# Autodesk Inventor assembly: rev6
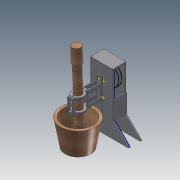
[picture p0: Inventor's stored thumbnail of the model, 180x180]
Saved by Autodesk Inventor 2015 (Build 190159000, 159)
## iProperties
Created: 2014-08-31
Part Number: rev6
Document SubType Name: Assembly
Designer: shohei
Author: shohei
## Documents named in this file (28)
- C:\Users\shohei\Documents\Inventor\FufuPounderGeared\rev6.iam
- C:\Users\shohei\Documents\Inventor\FufuPounderGeared\mortar2.ipt
- C:\Users\shohei\Documents\Inventor\FufuPounderGeared\sideplate.ipt
- C:\Users\shohei\Documents\Inventor\FufuPounderGeared\mainpulley.ipt
- C:\Users\shohei\Documents\Inventor\FufuPounderGeared\shaft5.ipt
- C:\Users\shohei\Documents\Inventor\FufuPounderGeared\drivelever.ipt
- C:\Users\shohei\Documents\Inventor\FufuPounderGeared\shaft7.ipt
- C:\Users\shohei\Documents\Inventor\FufuPounderGeared\globals.ipt
- C:\Users\shohei\Documents\Inventor\FufuPounderGeared\shaft8.ipt
- C:\Users\shohei\Documents\Inventor\FufuPounderGeared\shaft9.ipt
- C:\Users\shohei\Documents\Inventor\FufuPounderGeared\mallet_new.ipt
- C:\Users\shohei\Documents\Inventor\FufuPounderGeared\mallet_holder.ipt
- C:\Users\shohei\Documents\Inventor\FufuPounderGeared\mallet_sideplate.ipt
- C:\Users\shohei\Documents\Inventor\FufuPounderGeared\holderBlock.ipt
- C:\Users\shohei\Documents\Inventor\FufuPounderGeared\sideplate_top.ipt
- C:\Users\shohei\Documents\Inventor\FufuPounderGeared\shaft10.ipt
- C:\Users\shohei\Documents\Inventor\FufuPounderGeared\holderBlock2.ipt
- C:\Users\shohei\Documents\Inventor\FufuPounderGeared\gripsupport.ipt
- C:\Users\shohei\Documents\Inventor\FufuPounderGeared\M10washer.ipt
- C:\Users\shohei\Documents\Inventor\FufuPounderGeared\pulleyFlange.ipt
- C:\Users\shohei\Documents\Inventor\FufuPounderGeared\guardplate.ipt
- C:\Users\shohei\Documents\Inventor\FufuPounderGeared\drivepulleyAssembly.iam
- C:\Users\shohei\Documents\Inventor\FufuPounder\rev6\AIP\FEA\b5u4ebwdc.fins
- C:\Users\shohei\Documents\Inventor\FufuPounder\rev6\AIP\FEA\b5u4ebwdc.fsat
- C:\Users\shohei\Documents\Inventor\FufuPounder\rev6\AIP\FEA\b5u4ebwdc.ftes
- C:\Users\shohei\Documents\Inventor\FufuPounder\rev6\AIP\FEA\b5u4ebwdc.fwiz
- C:\Users\shohei\Documents\Inventor\FufuPounder\rev6\AIP\FEA\b5u4ebwgw.fmsh
- C:\Users\shohei\Documents\Inventor\FufuPounder\rev6\AIP\FEA\b5u4ebwgx.fres
## Components (46 placed, 21 different names)
1. mortar2:1 — Mate:1
2. sideplate:1 — Mate:2, Flush:1, Slider:1, Mate:9, Flush:13, Flush:14, Rotational:17, Flush:41, Mate:22
3. sideplate:2 — Mate:3, Flush:1, Rotational:10, Flush:15, Slider:2, Rotational:31, Mate:21, Flush:42
4. mainpulley:1 — Angle:1, Rotational:32, Cylindrical:6, Rigid:36, Rigid:38
5. shaft5:2 — Rotational:8, Cylindrical:6, Cylindrical:7
6. drivelever:1 — Cylindrical:1, Rotational:8, Rotational:23, Rotational:24, Rotational:25, Rotational:26
7. shaft7:1 — Slider:1, Cylindrical:1, Rotational:14, Rotational:18, Rotational:19, Rotational:20, Rotational:21
8. globals:1
9. mainpulley:2 — Cylindrical:7, Rotational:33, Rigid:35, Rigid:37
10. shaft8:1 — Rotational:10, Rotational:33
11. shaft9:2 — Cylindrical:4, Cylindrical:5, Slider:2, Rigid:2, Rotational:22
12. mallet_new:1 — Rigid:1
13. mallet_holder:1 — Flush:3, Mate:5, Flush:4, Mate:6, Flush:5, Flush:6, Flush:9, Mate:7, Flush:10, Mate:8, Flush:11, Flush:12, Rigid:1, Flush:32
14. mallet_holder:2 — Flush:7, Mate:15, Flush:29, Flush:37
15. mallet_sideplate:1 — Flush:3, Mate:5, Flush:4, Flush:7, Mate:15, Flush:34, Flush:35, Mate:18, Mate:19, Flush:38, Flush:39
16. mallet_sideplate:2 — Flush:9, Mate:7, Flush:10
17. mallet_sideplate:3 — Mate:6, Flush:5, Flush:6, Mate:16, Mate:17, Flush:33, Flush:36
18. mallet_sideplate:4 — Mate:8, Flush:11, Flush:12, Flush:37
19. holderBlock:2 — Rotational:14, Cylindrical:4
20. sideplate_top:1 — Mate:9, Flush:13, Flush:14, Flush:15
21. shaft10:1 — Rotational:17, Rotational:30, Rotational:32, Insert:1
22. holderBlock2:1 — Rotational:18, Cylindrical:5, Flush:28, Flush:40, Mate:20
23. gripsupport:1 — Flush:32, Mate:17, Flush:33, Flush:40
24. gripsupport:2 — Flush:34, Flush:35, Mate:18, Mate:20
25. gripsupport:3 — Mate:19, Flush:38, Flush:39
26. gripsupport:4 — Mate:16, Flush:28, Flush:29, Flush:36
27. pulleyFlange:1 — Rigid:36
28. pulleyFlange:2
29. pulleyFlange:3 — Rigid:35
30. guardplate:1 — Mate:22, Flush:42
31. guardplate:2 — Mate:21, Flush:41
32. drivepulleyAssembly:1 [sub-assembly] — Insert:1
33. M10washer:1 — Rigid:37
34. M10washer:2 — Rotational:19
35. M10washer:3 — Rotational:24
36. M10washer:4 — Rotational:25
37. M10washer:5 — Rotational:21
38. M10washer:6 — Rotational:22
39. M10washer:7 — Rotational:26
40. M10washer:8 — Rotational:23
41. M10washer:9 — Rotational:20
42. M10washer:10 — Rigid:2
43. M10washer:11 — Rigid:38
44. M10washer:14 — Rotational:31
45. M10washer:18 — Rotational:30
46. M10washer:22
## Relationships (74: Flush 26, RevoluteJoint 17, Mate 16, WeldJoint 6, CylindricalJoint 5, TranslationJoint 2, Angle 1, Insert 1)
- Mate:1: mortar2:1
- Mate:2: sideplate:1
- Mate:3: sideplate:2
- Flush:1: sideplate:1 ↔ sideplate:2
- Slider:1 [TranslationJoint]: sideplate:1 ↔ shaft7:1
- Cylindrical:1: drivelever:1 ↔ shaft7:1
- Rotational:8 [RevoluteJoint] (-30 mm): shaft5:2 ↔ drivelever:1
- Angle:1 (51.6389 deg): mainpulley:1
- Rotational:10 [RevoluteJoint]: sideplate:2 ↔ shaft8:1
- Flush:3: mallet_holder:1 ↔ mallet_sideplate:1
- Mate:5: mallet_holder:1 ↔ mallet_sideplate:1
- Flush:4: mallet_holder:1 ↔ mallet_sideplate:1
- Mate:6: mallet_holder:1 ↔ mallet_sideplate:3
- Flush:5: mallet_holder:1 ↔ mallet_sideplate:3
- Flush:6: mallet_holder:1 ↔ mallet_sideplate:3
- Flush:7: mallet_holder:2 ↔ mallet_sideplate:1
- Flush:9: mallet_holder:1 ↔ mallet_sideplate:2
- Mate:7: mallet_holder:1 ↔ mallet_sideplate:2
- Flush:10: mallet_holder:1 ↔ mallet_sideplate:2
- Mate:8: mallet_holder:1 ↔ mallet_sideplate:4
- Flush:11: mallet_holder:1 ↔ mallet_sideplate:4
- Flush:12: mallet_holder:1 ↔ mallet_sideplate:4
- Rotational:14 [RevoluteJoint] (-30 mm): shaft7:1 ↔ holderBlock:2
- Cylindrical:4: shaft9:2 ↔ holderBlock:2
- Mate:9: sideplate:1 ↔ sideplate_top:1
- Flush:13: sideplate:1 ↔ sideplate_top:1
- Flush:14: sideplate:1 ↔ sideplate_top:1
- Flush:15: sideplate:2 ↔ sideplate_top:1
- Rotational:17 [RevoluteJoint] (-80 mm): sideplate:1 ↔ shaft10:1
- Rotational:18 [RevoluteJoint]: shaft7:1 ↔ holderBlock2:1
- Cylindrical:5: shaft9:2 ↔ holderBlock2:1
- Mate:15: mallet_holder:2 ↔ mallet_sideplate:1
- Rigid:1 [WeldJoint]: mallet_new:1 ↔ mallet_holder:1
- Slider:2 [TranslationJoint]: sideplate:2 ↔ shaft9:2
- Mate:16: mallet_sideplate:3 ↔ gripsupport:4
- Flush:28: holderBlock2:1 ↔ gripsupport:4
- Flush:29: mallet_holder:2 ↔ gripsupport:4
- Rotational:19 [RevoluteJoint] (-22 mm): shaft7:1 ↔ M10washer:2
- Rotational:20 [RevoluteJoint] (-50 mm): shaft7:1 ↔ M10washer:9
- Rigid:2 [WeldJoint] (-20 mm): shaft9:2 ↔ M10washer:10
- Rotational:21 [RevoluteJoint] (-30 mm): shaft7:1 ↔ M10washer:5
- Rotational:22 [RevoluteJoint]: shaft9:2 ↔ M10washer:6
- Rotational:23 [RevoluteJoint] (-2 mm): drivelever:1 ↔ M10washer:8
- Rotational:24 [RevoluteJoint]: drivelever:1 ↔ M10washer:3
- Rotational:25 [RevoluteJoint]: drivelever:1 ↔ M10washer:4
- Rotational:26 [RevoluteJoint]: drivelever:1 ↔ M10washer:7
- Rotational:30 [RevoluteJoint] (-10 mm): shaft10:1 ↔ M10washer:18
- Rotational:31 [RevoluteJoint] (-2 mm): sideplate:2 ↔ M10washer:14
- Rotational:32 [RevoluteJoint]: mainpulley:1 ↔ shaft10:1
- Cylindrical:6: mainpulley:1 ↔ shaft5:2
- Cylindrical:7: shaft5:2 ↔ mainpulley:2
- Rotational:33 [RevoluteJoint] (10 mm): mainpulley:2 ↔ shaft8:1
- Rigid:35 [WeldJoint] (10 mm): mainpulley:2 ↔ pulleyFlange:3
- Rigid:36 [WeldJoint]: mainpulley:1 ↔ pulleyFlange:1
- Rigid:37 [WeldJoint]: mainpulley:2 ↔ M10washer:1
- Rigid:38 [WeldJoint]: mainpulley:1 ↔ M10washer:11
- Flush:32: mallet_holder:1 ↔ gripsupport:1
- Mate:17: mallet_sideplate:3 ↔ gripsupport:1
- Flush:33: mallet_sideplate:3 ↔ gripsupport:1
- Flush:34: mallet_sideplate:1 ↔ gripsupport:2
- Flush:35: mallet_sideplate:1 ↔ gripsupport:2
- Mate:18: mallet_sideplate:1 ↔ gripsupport:2
- Flush:36: mallet_sideplate:3 ↔ gripsupport:4
- Flush:37: mallet_holder:2 ↔ mallet_sideplate:4
- Mate:19: mallet_sideplate:1 ↔ gripsupport:3
- Flush:38: mallet_sideplate:1 ↔ gripsupport:3
- Flush:39: mallet_sideplate:1 ↔ gripsupport:3
- Flush:40: holderBlock2:1 ↔ gripsupport:1
- Mate:20: holderBlock2:1 ↔ gripsupport:2
- Mate:21: sideplate:2 ↔ guardplate:2
- Flush:41: sideplate:1 ↔ guardplate:2
- Mate:22: sideplate:1 ↔ guardplate:1
- Flush:42: sideplate:2 ↔ guardplate:1
- Insert:1: shaft10:1 ↔ drivepulleyAssembly:1
## Named parameters: sa_0 = 0, sa_1 = 3.2e-12, sa_2 = 10000
note: some values were not read from the file. Shown as the stored number, unit unknown: "sa_0", "sa_1", "sa_2".
